# Autodesk Inventor assembly: Сборка стенда
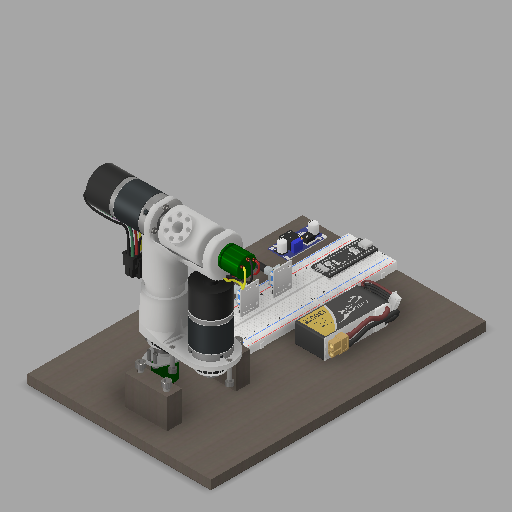
[picture p0: Inventor's stored thumbnail of the model, 512x512]
Saved by Autodesk Inventor 2025 (Build 290162000, 162)
## iProperties
Created: 2025-04-10
Part Number: Сборка стенда
Document SubType Name: Assembly
Designer: Artem Sannikov
Author: Artem Sannikov
## Documents named in this file (10)
- C:\Users\Artem Sannikov\Desktop\Two_axis_gimbal\3D_модели\Испытательный стенд\Сборка стенда.iam
- C:\Users\Artem Sannikov\Desktop\Two_axis_gimbal\3D_модели\Испытательный стенд\Основание.ipt
- C:\Users\Artem Sannikov\Desktop\Two_axis_gimbal\3D_модели\Основная сборка\Standard Large Breadboard with Two Side Rail.iam
- C:\Users\Artem Sannikov\Desktop\Two_axis_gimbal\3D_модели\Основная сборка\Black Pill.iam
- C:\Users\Artem Sannikov\Desktop\Two_axis_gimbal\3D_модели\Основная сборка\Основная сборка.iam
- C:\Users\Artem Sannikov\Desktop\Two_axis_gimbal\3D_модели\Испытательный стенд\Подставка.ipt
- C:\Users\Artem Sannikov\Documents\Inventor\Content Center Files\R2025\ru-RU\DIN 912\DIN 912 - M5 x 0,8 x 16 x 14.ipt
- C:\Users\Artem Sannikov\Desktop\Two_axis_gimbal\3D_модели\Испытательный стенд\TATTU 1300mah 3s.iam
- C:\Users\Artem Sannikov\Desktop\Two_axis_gimbal\3D_модели\Испытательный стенд\LM2596 DC-DC stepdown voltage converter.ipt
- C:\Users\Artem Sannikov\Desktop\Two_axis_gimbal\3D_модели\Испытательный стенд\rotary+encoder_17mm_hole_spc.ipt
## Components (13 placed, 9 different names)
1. Основание:1 — Совмещение:1, Заподлицо:1, Совмещение:5, Заподлицо:2, Совмещение:6, Заподлицо:3, Совмещение:8
2. Standard Large Breadboard with Two Side Rail:1 [sub-assembly] — Совмещение:1, Заподлицо:1, Совмещение:2, Совмещение:3, Совмещение:4, Совмещение:7, Заподлицо:3, Совмещение:9, Совмещение:10, Совмещение:11, Совмещение:12, Совмещение:13, Совмещение:14, Совмещение:15
3. Black Pill:1 [sub-assembly] — Совмещение:2, Совмещение:3, Совмещение:4
4. Основная сборка:1 [sub-assembly] — Совмещение:5, Вставка:1, Вставка:2, Вставка:3, Вставка:4
5. Подставка:1 — Заподлицо:2
6. DIN 912 - заменено на DIN EN ISO 4762 M5 x 16:1 — Вставка:1
7. DIN 912 - заменено на DIN EN ISO 4762 M5 x 16:2 — Вставка:2
8. DIN 912 - заменено на DIN EN ISO 4762 M5 x 16:3 — Вставка:3
9. DIN 912 - заменено на DIN EN ISO 4762 M5 x 16:4 — Вставка:4
10. TATTU 1300mah 3s:1 [sub-assembly] — Совмещение:6, Совмещение:7
11. LM2596 DC-DC stepdown voltage converter:1 — Совмещение:8, Совмещение:9
12. rotary+encoder_17mm_hole_spc:1 — Совмещение:10, Совмещение:11, Совмещение:12
13. rotary+encoder_17mm_hole_spc:2 — Совмещение:13, Совмещение:14, Совмещение:15
## Relationships (22: Mate 15, Insert 4, Flush 3)
- Совмещение:1 [Mate]: Основание:1 ↔ Standard Large Breadboard with Two Side Rail:1
- Заподлицо:1 [Flush]: Основание:1 ↔ Standard Large Breadboard with Two Side Rail:1
- Совмещение:2 [Mate]: Standard Large Breadboard with Two Side Rail:1 ↔ Black Pill:1
- Совмещение:3 [Mate]: Standard Large Breadboard with Two Side Rail:1 ↔ Black Pill:1
- Совмещение:4 [Mate]: Standard Large Breadboard with Two Side Rail:1 ↔ Black Pill:1
- Совмещение:5 [Mate] (5 mm): Основание:1 ↔ Основная сборка:1
- Заподлицо:2 [Flush]: Основание:1 ↔ Подставка:1
- Вставка:1 [Insert]: Основная сборка:1 ↔ DIN 912 - заменено на DIN EN ISO 4762 M5 x 16:1
- Вставка:2 [Insert]: Основная сборка:1 ↔ DIN 912 - заменено на DIN EN ISO 4762 M5 x 16:2
- Вставка:3 [Insert]: Основная сборка:1 ↔ DIN 912 - заменено на DIN EN ISO 4762 M5 x 16:3
- Вставка:4 [Insert]: Основная сборка:1 ↔ DIN 912 - заменено на DIN EN ISO 4762 M5 x 16:4
- Совмещение:6 [Mate]: Основание:1 ↔ TATTU 1300mah 3s:1
- Совмещение:7 [Mate] (15 mm): Standard Large Breadboard with Two Side Rail:1 ↔ TATTU 1300mah 3s:1
- Заподлицо:3 [Flush] (50 mm): Основание:1 ↔ Standard Large Breadboard with Two Side Rail:1
- Совмещение:8 [Mate]: Основание:1 ↔ LM2596 DC-DC stepdown voltage converter:1
- Совмещение:9 [Mate] (15 mm): Standard Large Breadboard with Two Side Rail:1 ↔ LM2596 DC-DC stepdown voltage converter:1
- Совмещение:10 [Mate]: Standard Large Breadboard with Two Side Rail:1 ↔ rotary+encoder_17mm_hole_spc:1
- Совмещение:11 [Mate]: Standard Large Breadboard with Two Side Rail:1 ↔ rotary+encoder_17mm_hole_spc:1
- Совмещение:12 [Mate]: Standard Large Breadboard with Two Side Rail:1 ↔ rotary+encoder_17mm_hole_spc:1
- Совмещение:13 [Mate]: Standard Large Breadboard with Two Side Rail:1 ↔ rotary+encoder_17mm_hole_spc:2
- Совмещение:14 [Mate]: Standard Large Breadboard with Two Side Rail:1 ↔ rotary+encoder_17mm_hole_spc:2
- Совмещение:15 [Mate]: Standard Large Breadboard with Two Side Rail:1 ↔ rotary+encoder_17mm_hole_spc:2
